# Autodesk Inventor assembly: Elevator MK2
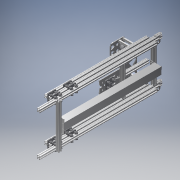
[picture p0: Inventor's stored thumbnail of the model, 180x180]
Saved by Autodesk Inventor 2019.4 (Build 234330000, 330)
## iProperties
Created: 2020-01-23
Part Number: Elevator MK2
Document SubType Name: Assembly
Designer: Mark
Mass: 5797.54 g
Surface Area: 14704.9 cm^2
Volume: 2466.95 cm^3
Density: 2.35008 g/cm^3
Author: Mark
## Documents named in this file (16)
- C:\Users\Mark\Desktop\7738 Helion Engineering\7738-2020\Elevator MK2\Elevator MK2.iam
- C:\Users\Mark\Desktop\7738 Helion Engineering\7738-2020\Spinny disk assembly\Aluminium extrusion profile 2020.ipt
- C:\Users\Mark\Desktop\7738 Helion Engineering\7738-2020\Elevator MK2\Mini V Gantry Kit.ipt
- C:\Users\Mark\Desktop\7738 Helion Engineering\7738-2020\Elevator MK2\Second Stage  Extrusion.ipt
- C:\Users\Mark\Desktop\7738 Helion Engineering\7738-2020\Elevator MK2\Final Stage.ipt
- C:\Users\Mark\Desktop\7738 Helion Engineering\7738-2020\Elevator MK2\Final Extrusion Mid.ipt
- **C:\Users\Mark\Desktop\7738 Helion Engineering\7738-2020\Robot Assembly MK2.iam*LocalDocs*x2tom4pch4vblelovMqgcvgtxXa*AdjusterAssembly.iam
- C:\Users\Mark\Desktop\7738 Helion Engineering\7738-2020\Elevator MK2\Up extrusion.ipt
- C:\Users\Mark\Desktop\7738 Helion Engineering\7738-2020\Elevator MK2\M6 Eye Bolt.ipt
- C:\Users\Mark\Desktop\7738 Helion Engineering\7738-2020\Elevator MK2\Pulley plate.ipt
- C:\Users\Mark\Desktop\7738 Helion Engineering\7738-2020\Elevator MK2\608 Bearing.ipt
- C:\Users\Mark\Desktop\7738 Helion Engineering\7738-2020\Elevator MK2\SC32-600.ipt
- C:\Users\Mark\Desktop\7738 Helion Engineering\7738-2020\Elevator MK2\SC32 Bore.ipt
- C:\Users\Mark\Desktop\7738 Helion Engineering\7738-2020\Elevator MK2\Bottom Pneumatic Extrusion.ipt
- C:\Users\Mark\Desktop\7738 Helion Engineering\7738-2020\Elevator MK2\Pneumatic Bottom Plate.ipt
- C:\Users\Mark\Desktop\7738 Helion Engineering\7738-2020\Elevator MK2\Top Plate.ipt
## Components (31 placed, 15 different names)
1. Aluminium extrusion profile 2020:1 — Flush:1, Flush:2, Mate:1, Flush:17, Mate:45, Mate:46
2. Aluminium extrusion profile 2020:2 — Flush:1, Flush:2, Mate:1, Mate:23, Mate:43, Mate:44, Flush:48, Mate:66, Flush:49
3. Mini V Gantry Kit:1 — Mate:12, Mate:13, Mate:14
4. Mini V Gantry Kit:2 — Mate:27, Mate:28, Mate:29
5. Mini V Gantry Kit:3 — Mate:24, Mate:25, Mate:26
6. Mini V Gantry Kit:4 — Mate:15, Mate:16, Mate:17
7. Second Stage  Extrusion:1 — Mate:12, Mate:13, Mate:14, Mate:15, Mate:16, Mate:17, Flush:17, Mate:19, Flush:18, Flush:19, Mate:54, Flush:32, Mate:55
8. Second Stage  Extrusion:2 — Mate:19, Flush:18, Flush:19, Mate:20, Mate:21, Mate:22, Mate:23, Flush:23, Mate:37, Mate:59, Mate:60, Flush:35, Flush:45, Mate:67, Flush:50, Flush:51
9. Final Stage:1 — Mate:24, Mate:25, Mate:26, Mate:27, Mate:28, Mate:29, Flush:21, Flush:22, Flush:23, Mate:37, Mate:38, Mate:39, Flush:25, Mate:41, Flush:45, Flush:47
10. Mini V Gantry Kit:5 — Mate:20, Mate:21, Mate:22
11. Mini V Gantry Kit:8
12. Mini V Gantry Kit:9
13. Mini V Gantry Kit:10
14. Final Stage:2 — Flush:21, Flush:22, Mate:38, Flush:28
15. Final Extrusion Mid:1 — Mate:39, Flush:25, Mate:40, Flush:26, Flush:28
16. AdjusterAssembly:1 [sub-assembly] — Mate:65, Flush:46, Flush:47
17. Up extrusion:1 — Mate:40, Flush:26, Mate:41, Mate:65, Flush:46
18. M6 Eye Bolt:1 — Mate:43, Mate:44, Flush:29
19. M6 Eye Bolt:2 — Mate:45, Mate:46, Flush:29
20. Pulley plate:1 — Flush:30, Mate:51, Mate:52, Flush:31, Mate:54, Flush:32, Mate:55
21. Pulley plate:2 — Flush:30, Mate:51, Mate:53, Flush:31
22. 608 Bearing:1 — Mate:52, Mate:53
23. Pulley plate:3 — Mate:59, Mate:60, Flush:35
24. Pulley plate:4
25. 608 Bearing:2
26. SC32-600:1 — Elevator, Mate:68, Flush:52, Flush:53
27. SC32 Bore:1 — Elevator, Mate:70, Mate:71
28. Bottom Pneumatic Extrusion:1 — Flush:48, Mate:66, Flush:49, Mate:69, Flush:54, Flush:55
29. Final Extrusion Mid:2 — Mate:67, Flush:50, Flush:51, Mate:70, Mate:72, Flush:56
30. Pneumatic Bottom Plate:1 — Mate:68, Flush:52, Flush:53, Mate:69, Flush:54, Flush:55
31. Top Plate:1 — Mate:71, Mate:72, Flush:56
## Relationships (85: Mate 52, Flush 32, CylindricalJoint 1)
- Flush:1: Aluminium extrusion profile 2020:1 ↔ Aluminium extrusion profile 2020:2
- Flush:2: Aluminium extrusion profile 2020:1 ↔ Aluminium extrusion profile 2020:2
- Mate:1 (239 mm): Aluminium extrusion profile 2020:1 ↔ Aluminium extrusion profile 2020:2
- [Flush]: Mini V Gantry Kit:5 ↔ Mini V Gantry Kit:8
- [Flush]: Mini V Gantry Kit:5 ↔ Mini V Gantry Kit:8
- [Mate] (50 mm): Mini V Gantry Kit:5 ↔ Mini V Gantry Kit:8
- Mate:12: Mini V Gantry Kit:1 ↔ Second Stage  Extrusion:1
- Mate:13: Mini V Gantry Kit:1 ↔ Second Stage  Extrusion:1
- Mate:14: Mini V Gantry Kit:1 ↔ Second Stage  Extrusion:1
- Mate:15: Mini V Gantry Kit:4 ↔ Second Stage  Extrusion:1
- Mate:16: Mini V Gantry Kit:4 ↔ Second Stage  Extrusion:1
- Mate:17: Mini V Gantry Kit:4 ↔ Second Stage  Extrusion:1
- Flush:17: Aluminium extrusion profile 2020:1 ↔ Second Stage  Extrusion:1
- Mate:19 (239 mm): Second Stage  Extrusion:1 ↔ Second Stage  Extrusion:2
- Flush:18: Second Stage  Extrusion:1 ↔ Second Stage  Extrusion:2
- Flush:19: Second Stage  Extrusion:1 ↔ Second Stage  Extrusion:2
- Mate:20: Second Stage  Extrusion:2 ↔ Mini V Gantry Kit:5
- Mate:21: Second Stage  Extrusion:2 ↔ Mini V Gantry Kit:5
- Mate:22: Second Stage  Extrusion:2 ↔ Mini V Gantry Kit:5
- Mate:23 (6.4 mm): Aluminium extrusion profile 2020:2 ↔ Second Stage  Extrusion:2
- Mate:24: Mini V Gantry Kit:3 ↔ Final Stage:1
- Mate:25: Mini V Gantry Kit:3 ↔ Final Stage:1
- Mate:26: Mini V Gantry Kit:3 ↔ Final Stage:1
- Mate:27: Mini V Gantry Kit:2 ↔ Final Stage:1
- Mate:28: Mini V Gantry Kit:2 ↔ Final Stage:1
- Mate:29: Mini V Gantry Kit:2 ↔ Final Stage:1
- [Mate]: Mini V Gantry Kit:10 ↔ Final Stage:2
- [Mate]: Mini V Gantry Kit:10 ↔ Final Stage:2
- [Mate]: Mini V Gantry Kit:10 ↔ Final Stage:2
- [Mate]: Mini V Gantry Kit:9 ↔ Final Stage:2
- [Mate]: Mini V Gantry Kit:9 ↔ Final Stage:2
- [Mate]: Mini V Gantry Kit:9 ↔ Final Stage:2
- Flush:21: Final Stage:1 ↔ Final Stage:2
- Flush:22: Final Stage:1 ↔ Final Stage:2
- Flush:23: Second Stage  Extrusion:2 ↔ Final Stage:1
- Mate:37 (6.4 mm): Second Stage  Extrusion:2 ↔ Final Stage:1
- Mate:38 (239 mm): Final Stage:1 ↔ Final Stage:2
- Mate:39: Final Stage:1 ↔ Final Extrusion Mid:1
- Flush:25: Final Stage:1 ↔ Final Extrusion Mid:1
- Mate:40: Final Extrusion Mid:1 ↔ Up extrusion:1
- Flush:26: Final Extrusion Mid:1 ↔ Up extrusion:1
- Mate:41 (114.5 mm): Final Stage:1 ↔ Up extrusion:1
- Flush:28 (150 mm): Final Stage:2 ↔ Final Extrusion Mid:1
- Mate:43: Aluminium extrusion profile 2020:2 ↔ M6 Eye Bolt:1
- Mate:44: Aluminium extrusion profile 2020:2 ↔ M6 Eye Bolt:1
- Mate:45: Aluminium extrusion profile 2020:1 ↔ M6 Eye Bolt:2
- Mate:46: Aluminium extrusion profile 2020:1 ↔ M6 Eye Bolt:2
- Flush:29: M6 Eye Bolt:1 ↔ M6 Eye Bolt:2
- Flush:30: Pulley plate:1 ↔ Pulley plate:2
- Mate:51 (20 mm): Pulley plate:1 ↔ Pulley plate:2
- Mate:52: Pulley plate:1 ↔ 608 Bearing:1
- Mate:53 (6.5 mm): Pulley plate:2 ↔ 608 Bearing:1
- Flush:31: Pulley plate:1 ↔ Pulley plate:2
- Mate:54: Second Stage  Extrusion:1 ↔ Pulley plate:1
- Flush:32: Second Stage  Extrusion:1 ↔ Pulley plate:1
- Mate:55 (-19 mm): Second Stage  Extrusion:1 ↔ Pulley plate:1
- [Flush]: Pulley plate:3 ↔ Pulley plate:4
- [Mate] (20 mm): Pulley plate:3 ↔ Pulley plate:4
- [Mate]: Pulley plate:3 ↔ 608 Bearing:2
- [Mate] (6.5 mm): Pulley plate:4 ↔ 608 Bearing:2
- [Flush]: Pulley plate:3 ↔ Pulley plate:4
- Mate:59: Second Stage  Extrusion:2 ↔ Pulley plate:3
- Mate:60 (-19 mm): Second Stage  Extrusion:2 ↔ Pulley plate:3
- Flush:35: Second Stage  Extrusion:2 ↔ Pulley plate:3
- Elevator [CylindricalJoint]: SC32-600:1 ↔ SC32 Bore:1
- Flush:45: Second Stage  Extrusion:2 ↔ Final Stage:1
- Mate:65 (0.4 mm): AdjusterAssembly:1 ↔ Up extrusion:1
- Flush:46 (-15 mm): AdjusterAssembly:1 ↔ Up extrusion:1
- Flush:47: Final Stage:1 ↔ AdjusterAssembly:1
- Flush:48: Aluminium extrusion profile 2020:2 ↔ Bottom Pneumatic Extrusion:1
- Mate:66: Aluminium extrusion profile 2020:2 ↔ Bottom Pneumatic Extrusion:1
- Flush:49 (100 mm): Aluminium extrusion profile 2020:2 ↔ Bottom Pneumatic Extrusion:1
- Mate:67: Second Stage  Extrusion:2 ↔ Final Extrusion Mid:2
- Flush:50: Second Stage  Extrusion:2 ↔ Final Extrusion Mid:2
- Flush:51 (19 mm): Second Stage  Extrusion:2 ↔ Final Extrusion Mid:2
- Mate:68: SC32-600:1 ↔ Pneumatic Bottom Plate:1
- Flush:52: SC32-600:1 ↔ Pneumatic Bottom Plate:1
- Flush:53 (-20 mm): SC32-600:1 ↔ Pneumatic Bottom Plate:1
- Mate:69: Bottom Pneumatic Extrusion:1 ↔ Pneumatic Bottom Plate:1
- Flush:54 (-12.5 mm): Bottom Pneumatic Extrusion:1 ↔ Pneumatic Bottom Plate:1
- Flush:55 (97 mm): Bottom Pneumatic Extrusion:1 ↔ Pneumatic Bottom Plate:1
- Mate:70 (-12 mm): SC32 Bore:1 ↔ Final Extrusion Mid:2
- Mate:71: SC32 Bore:1 ↔ Top Plate:1
- Mate:72: Final Extrusion Mid:2 ↔ Top Plate:1
- Flush:56: Final Extrusion Mid:2 ↔ Top Plate:1
## Named parameters: d22_d13 = 50 mm, d25_d48 = 0 mm, d26_d49 = 0 mm, d51_d45 = 0 mm, d52_d46 = 0 mm, d53_d47 = 0 mm, d54_d48 = 0 mm, d55_d49 = 0 mm, d56_d50 = 0 mm, d98_d92 = 0 mm, d99_d93 = 6.5 mm, d100_d94 = 0 mm, d101_d90 = 0 mm, d102_d91 = 20 mm, ElevatorPosition = 22 mm
